# Autodesk Inventor assembly: MotorMountAssembly
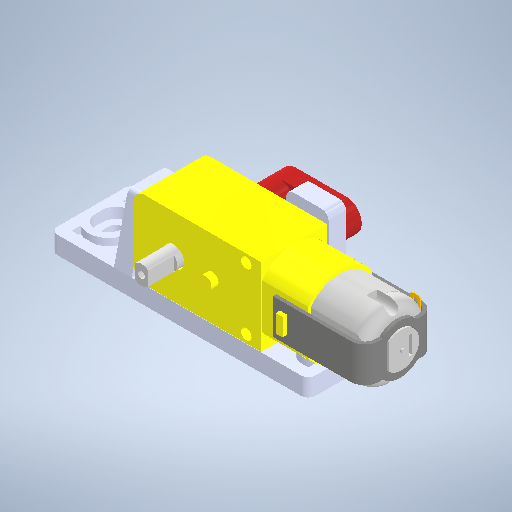
[picture p0: Inventor's stored thumbnail of the model, 512x512]
Saved by Autodesk Inventor 2026 (Build 300175050, 175E)
## iProperties
Created: 2025-06-11
Part Number: MotorMountAssembly
Document SubType Name: Assembly
Designer: omiye
Author: omiye
## Documents named in this file (4)
- C:\Projects\Arduino\strandbeest\MotorMountAssembly.iam
- C:\Projects\Arduino\strandbeest\6VDC_motor_mount_REV2.ipt
- C:\Projects\Arduino\strandbeest\yellow_toy_motor_dims.ipt
- C:\Projects\Arduino\strandbeest\newM.ipt
## Components (3 placed, 3 different names)
1. 6VDC_motor_mount_REV2:1 — Mate:1, Mate:2, Mate:3
2. yellow_toy_motor_dims:1 — Mate:1, Mate:2, Mate:3, Mate:4, Mate:5
3. newM:1 — Mate:4, Mate:5
## Relationships (5: Mate 5)
- Mate:1: 6VDC_motor_mount_REV2:1 ↔ yellow_toy_motor_dims:1
- Mate:2: 6VDC_motor_mount_REV2:1 ↔ yellow_toy_motor_dims:1
- Mate:3: 6VDC_motor_mount_REV2:1 ↔ yellow_toy_motor_dims:1
- Mate:4: yellow_toy_motor_dims:1 ↔ newM:1
- Mate:5: yellow_toy_motor_dims:1 ↔ newM:1
